# Autodesk Inventor assembly: LongboardBare
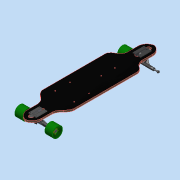
[picture p0: Inventor's stored thumbnail of the model, 180x180]
Saved by Autodesk Inventor 2015 SP1 (Build 190203100, 203)
## iProperties
Created: 2015-06-13
Part Number: LongboardBare
Document SubType Name: Assembly
Designer: YOUR_NAME_HERE
Author: YOUR_NAME_HERE
## Documents named in this file (4)
- C:\Users\Rahul\Electric Skateboard\Electric Skateboard CAD\LongboardBare.iam
- C:\Users\Rahul\Electric Skateboard\Electric Skateboard CAD\LongboardDeck.ipt
- C:\Users\Rahul\Electric Skateboard\Electric Skateboard CAD\suspension_assy.iam
- C:\Users\Rahul\Electric Skateboard\Electric Skateboard CAD\suspension_assy_normal.iam
## Components (3 placed, 3 different names)
1. LongboardDeck:1 — Mate:3, Mate:4, Mate:5, Mate:6, Mate:7, Flush:1
2. suspension_assy:2 [sub-assembly] — Mate:3, Mate:4, Mate:5
3. suspension_assy_normal:1 [sub-assembly] — Mate:6, Mate:7, Flush:1
## Relationships (6: Mate 5, Flush 1)
- Mate:3: LongboardDeck:1 ↔ suspension_assy:2
- Mate:4: LongboardDeck:1 ↔ suspension_assy:2
- Mate:5 (47.625 mm): LongboardDeck:1 ↔ suspension_assy:2
- Mate:6: LongboardDeck:1 ↔ suspension_assy_normal:1
- Mate:7: LongboardDeck:1 ↔ suspension_assy_normal:1
- Flush:1 (47.625 mm): LongboardDeck:1 ↔ suspension_assy_normal:1
